# Autodesk Inventor assembly: BREEZE-S01
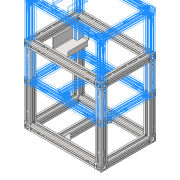
[picture p0: Inventor's stored thumbnail of the model, 180x180]
Saved by Autodesk Inventor 2020 (Build 240168000, 168)
## iProperties
Created: 2020-04-12
Part Number: BREEZE-S01
Document SubType Name: Assembly
Designer: John K
Description: FRAME ASSEMBLY
Author: John K
## Documents named in this file (9)
- C:\GrabCAD\MTL Ventilator Design\BREEZE\Subassemblies\BREEZE-S01.iam
- C:\GrabCAD\MTL Ventilator Design\BREEZE\Manufactured Parts\BREEZE-M01.ipt
- C:\GrabCAD\MTL Ventilator Design\BREEZE\Manufactured Parts\BREEZE-M03.ipt
- C:\GrabCAD\MTL Ventilator Design\BREEZE\Commercial Parts\McMaster\Frame Corner.ipt
- C:\GrabCAD\MTL Ventilator Design\BREEZE\Commercial Parts\McMaster\Frame Bracket.ipt
- C:\GrabCAD\MTL Ventilator Design\BREEZE\Manufactured Parts\BREEZE-M04.ipt
- C:\GrabCAD\MTL Ventilator Design\BREEZE\Commercial Parts\McMaster\M5x14mm Button.ipt
- C:\GrabCAD\MTL Ventilator Design\BREEZE\Commercial Parts\McMaster\M5 T-Slot Fastener.ipt
- C:\GrabCAD\MTL Ventilator Design\BREEZE\Commercial Parts\McMaster\M5x8mm Flanged Button.ipt
## Components (104 placed, 8 different names)
1. BREEZE-M01:1 — Flush:1, Flush:2, Flush:3, Flush:4, Symmetry:1, Symmetry:2, Mate:1, Mate:2, Flush:10, Mate:3, Mate:4, Mate:5, Mate:6, Mate:7, Flush:24, Mate:10, Mate:14, Flush:74, Flush:117
2. BREEZE-M01:2 — Flush:2, Symmetry:2, Flush:5, Mate:2, Flush:26
3. BREEZE-M01:3 — Flush:3, Flush:5, Flush:6, Mate:22, Mate:24
4. BREEZE-M01:4 — Flush:4, Symmetry:1, Mate:1, Flush:6, Flush:11, Mate:8, Mate:23, Mate:25, Mate:26
5. BREEZE-M01:5 — Flush:7, Flush:8, Flush:9, Flush:10, Mate:3, Mate:4, Flush:12, Flush:13, Flush:14, Flush:25, Mate:15, Mate:17, Mate:19, Mate:43
6. BREEZE-M01:6 — Flush:7, Flush:9, Flush:11, Flush:16, Mate:20, Flush:71, Mate:40, Flush:100
7. BREEZE-M01:7 — Flush:12, Flush:13, Flush:15, Mate:5, Mate:11, Mate:13, Flush:49, Flush:85, Mate:34, Mate:36, Flush:112
8. BREEZE-M01:8 — Flush:14, Flush:15, Flush:16, Flush:70, Flush:86, Flush:113
9. BREEZE-M03:1 — Flush:17, Flush:18, Flush:19, Flush:21, Flush:23, Mate:6, Mate:7, Flush:24, Mate:8, Mate:9, Mate:12, Mate:30, Flush:84, Mate:32
10. BREEZE-M03:2 — Flush:17, Flush:21, Flush:22, Flush:26, Mate:21, Flush:48, Mate:31, Flush:88, Flush:87, Flush:93, Flush:94, Mate:37, Flush:89
11. BREEZE-M03:3 — Flush:19, Flush:20, Flush:22, Flush:47
12. BREEZE-M03:4 — Flush:18, Flush:20, Flush:23, Flush:25, Mate:16, Flush:43
13. BREEZE-M03:5 — Flush:43, Mate:17, Flush:45, Mate:18, Flush:47, Mate:38, Mate:39
14. BREEZE-M04:1 — Mate:21, Flush:48, Flush:49
15. Frame Corner:1 — Mate:9, Mate:10, Mate:11, Flush:27, Flush:28, Flush:29, Flush:30, Flush:33, Flush:34, Flush:35, Insert:1, Insert:2, Insert:3
16. Frame Corner:2 — Flush:27, Flush:30, Flush:31, Mate:13, Insert:4, Insert:5, Insert:6
17. Frame Corner:3 — Flush:29, Flush:31, Flush:32, Insert:7, Insert:8, Insert:9
18. Frame Corner:4 — Flush:28, Flush:32, Flush:33, Mate:12, Insert:10, Insert:11, Insert:12
19. Frame Corner:5 — Flush:34, Flush:35, Mate:14, Flush:36, Flush:37, Flush:39, Flush:40, Flush:42, Insert:13, Insert:14, Insert:15
20. Frame Corner:6 — Flush:36, Flush:37, Mate:15, Flush:38, Insert:16, Insert:17, Insert:18
21. Frame Corner:7 — Flush:38, Flush:39, Flush:41, Insert:19, Insert:20, Insert:21
22. Frame Corner:8 — Flush:40, Flush:41, Flush:42, Mate:16, Insert:22, Insert:23, Insert:24
23. Frame Bracket:1 — Flush:44, Flush:45, Flush:46, Mate:18, Mate:20, Mate:41, Mate:42
24. Frame Bracket:2 — Flush:44, Flush:46, Mate:19
25. M5 T-Slot Fastener:48 — Flush:112, Flush:114, Flush:115, Flush:116, Flush:117
26. M5 T-Slot Fastener:49 — Flush:113, Flush:114, Flush:115
27. M5x14mm Button:1 — Insert:1
28. M5x14mm Button:2 — Insert:2
29. M5x14mm Button:3 — Insert:3
30. M5x14mm Button:4 — Insert:4
31. M5x14mm Button:5 — Insert:5
32. M5x14mm Button:6 — Insert:6
33. M5x14mm Button:7 — Insert:7
34. M5x14mm Button:8 — Insert:8
35. M5x14mm Button:9 — Insert:9
36. M5x14mm Button:10 — Insert:10
37. M5x14mm Button:11 — Insert:11
38. M5x14mm Button:12 — Insert:12
39. M5x14mm Button:13 — Insert:13
40. M5x14mm Button:14 — Insert:14
41. M5x14mm Button:15 — Insert:15
42. M5x14mm Button:16 — Insert:16
43. M5x14mm Button:17 — Insert:17
44. M5x14mm Button:18 — Insert:18
45. M5x14mm Button:19 — Insert:19
46. M5x14mm Button:20 — Insert:20
47. M5x14mm Button:21 — Insert:21
48. M5x14mm Button:22 — Insert:22
49. M5x14mm Button:23 — Insert:23
50. M5x14mm Button:24 — Insert:24
51. M5 T-Slot Fastener:37 — Flush:90, Flush:91, Flush:92, Mate:33, Flush:93, Mate:35, Flush:94, Mate:37, Insert:25
52. M5 T-Slot Fastener:38 — Flush:90, Mate:34, Mate:36, Insert:27, Flush:116
53. M5 T-Slot Fastener:39 — Flush:91, Flush:92, Mate:33, Mate:35, Insert:26
54. M5x8mm Flanged Button:1 — Insert:25
55. M5x8mm Flanged Button:2 — Insert:26
56. M5x8mm Flanged Button:3 — Insert:27
57. M5 T-Slot Fastener:40 — Flush:98, Mate:43, Flush:99, Insert:28
58. M5 T-Slot Fastener:41 — Flush:95, Flush:96, Symmetry:6, Insert:29
59. M5 T-Slot Fastener:42 — Flush:95, Flush:96, Flush:97, Flush:98, Mate:38, Symmetry:6, Mate:39, Mate:42, Insert:30
60. M5 T-Slot Fastener:43 — Flush:97, Mate:40, Mate:41, Flush:99, Insert:31
61. M5x8mm Flanged Button:4 — Insert:28
62. M5x8mm Flanged Button:5 — Insert:29
63. M5x8mm Flanged Button:6 — Insert:30
64. M5x8mm Flanged Button:7 — Insert:31
65. M5 T-Slot Fastener:44 — Flush:101, Flush:102, Flush:111
66. M5 T-Slot Fastener:45 — Flush:103, Flush:104, Flush:110
67. M5 T-Slot Fastener:46 — Flush:105, Flush:107, Mate:44, Flush:111
68. M5 T-Slot Fastener:47 — Flush:106, Flush:108, Flush:109, Flush:110
69. M5 T-Slot Fastener:1 — Flush:55, Flush:61, Flush:65, Flush:66, Mate:22, Mate:24, Flush:87
70. M5 T-Slot Fastener:12 — Flush:64, Flush:65, Flush:69, Flush:70, Flush:88, Symmetry:4
71. M5 T-Slot Fastener:9 — Flush:60, Flush:64, Flush:68, Symmetry:4
72. M5 T-Slot Fastener:2 — Flush:59, Flush:60, Flush:63, Flush:66, Mate:23, Flush:75
73. M5 T-Slot Fastener:8 — Flush:58, Flush:59, Flush:63, Flush:67, Flush:76
74. M5 T-Slot Fastener:10 — Flush:57, Flush:58, Flush:62, Flush:68
75. M5 T-Slot Fastener:11 — Flush:56, Flush:57, Flush:62, Flush:69, Flush:71
76. M5 T-Slot Fastener:7 — Flush:55, Flush:56, Flush:61, Flush:67, Flush:100
77. M5 T-Slot Fastener:3 — Flush:50, Flush:54, Flush:72, Mate:25, Mate:26, Flush:75
78. M5 T-Slot Fastener:4 — Flush:52, Flush:53, Flush:72, Flush:74
79. M5 T-Slot Fastener:6 — Flush:51, Flush:52, Flush:53, Flush:73
80. M5 T-Slot Fastener:5 — Flush:50, Flush:51, Flush:54, Flush:73, Flush:76
81. M5 T-Slot Fastener:19
82. M5 T-Slot Fastener:20
83. M5 T-Slot Fastener:21
84. M5 T-Slot Fastener:22
85. M5 T-Slot Fastener:23
86. M5 T-Slot Fastener:24
87. M5 T-Slot Fastener:25
88. M5 T-Slot Fastener:26
89. M5 T-Slot Fastener:27
90. M5 T-Slot Fastener:28
91. M5 T-Slot Fastener:29
92. M5 T-Slot Fastener:30
93. M5 T-Slot Fastener:14 — Flush:78, Flush:79, Mate:28, Flush:82, Flush:89, Symmetry:5
94. M5 T-Slot Fastener:16 — Flush:79, Flush:80, Mate:28, Flush:83, Flush:86, Symmetry:5
95. M5 T-Slot Fastener:17 — Flush:81, Mate:27, Flush:83, Flush:85
96. M5 T-Slot Fastener:15 — Flush:77, Flush:78, Mate:29, Mate:30, Flush:84, Mate:32, Flush:105, Flush:106, Flush:107, Flush:108, Flush:109, Mate:44
97. M5 T-Slot Fastener:13 — Flush:77, Mate:27, Flush:82
98. M5 T-Slot Fastener:18 — Flush:80, Flush:81, Mate:29, Mate:31, Flush:101, Flush:102, Flush:103, Flush:104
99. M5 T-Slot Fastener:31
100. M5 T-Slot Fastener:32
101. M5 T-Slot Fastener:33
102. M5 T-Slot Fastener:34
103. M5 T-Slot Fastener:35
104. M5 T-Slot Fastener:36
## Component patterns: (2 elements, first: M5 T-Slot Fastener:1 + M5 T-Slot Fastener:12 + M5 T-Slot Fastener:9 + M5 T-Slot Fastener:2 + M5 T-Slot Fastener:8 + M5 T-Slot Fastener:10 + M5 T-Slot Fastener:11 + M5 T-Slot Fastener:7 + M5 T-Slot Fastener:3 + M5 T-Slot Fastener:4 + M5 T-Slot Fastener:6 + M5 T-Slot Fastener:5), (2 elements, first: M5 T-Slot Fastener:14 + M5 T-Slot Fastener:16 + M5 T-Slot Fastener:17 + M5 T-Slot Fastener:15 + M5 T-Slot Fastener:13 + M5 T-Slot Fastener:18)
## Relationships (197: Flush 117, Mate 44, Insert 31, Symmetry 5)
- Flush:1: BREEZE-M01:1
- Flush:2: BREEZE-M01:1 ↔ BREEZE-M01:2
- Flush:3: BREEZE-M01:1 ↔ BREEZE-M01:3
- Flush:4: BREEZE-M01:1 ↔ BREEZE-M01:4
- Symmetry:1: BREEZE-M01:1 ↔ BREEZE-M01:4
- Symmetry:2: BREEZE-M01:1 ↔ BREEZE-M01:2
- Mate:1: BREEZE-M01:1 ↔ BREEZE-M01:4
- Flush:5: BREEZE-M01:2 ↔ BREEZE-M01:3
- Mate:2: BREEZE-M01:1 ↔ BREEZE-M01:2
- Flush:6: BREEZE-M01:3 ↔ BREEZE-M01:4
- Flush:7: BREEZE-M01:5 ↔ BREEZE-M01:6
- Flush:8: BREEZE-M01:5
- Flush:9: BREEZE-M01:5 ↔ BREEZE-M01:6
- Flush:10: BREEZE-M01:1 ↔ BREEZE-M01:5
- Flush:11: BREEZE-M01:4 ↔ BREEZE-M01:6
- Mate:3: BREEZE-M01:1 ↔ BREEZE-M01:5
- Mate:4: BREEZE-M01:1 ↔ BREEZE-M01:5
- Flush:12: BREEZE-M01:5 ↔ BREEZE-M01:7
- Flush:13: BREEZE-M01:5 ↔ BREEZE-M01:7
- Flush:14: BREEZE-M01:5 ↔ BREEZE-M01:8
- Flush:15: BREEZE-M01:7 ↔ BREEZE-M01:8
- Mate:5: BREEZE-M01:1 ↔ BREEZE-M01:7
- Flush:16: BREEZE-M01:6 ↔ BREEZE-M01:8
- Flush:17: BREEZE-M03:1 ↔ BREEZE-M03:2
- Flush:18: BREEZE-M03:1 ↔ BREEZE-M03:4
- Flush:19: BREEZE-M03:1 ↔ BREEZE-M03:3
- Flush:20: BREEZE-M03:3 ↔ BREEZE-M03:4
- Flush:21: BREEZE-M03:1 ↔ BREEZE-M03:2
- Flush:22: BREEZE-M03:2 ↔ BREEZE-M03:3
- Flush:23: BREEZE-M03:1 ↔ BREEZE-M03:4
- Mate:6: BREEZE-M01:1 ↔ BREEZE-M03:1
- Mate:7: BREEZE-M01:1 ↔ BREEZE-M03:1
- Flush:24: BREEZE-M01:1 ↔ BREEZE-M03:1
- Flush:25: BREEZE-M01:5 ↔ BREEZE-M03:4
- Flush:26: BREEZE-M01:2 ↔ BREEZE-M03:2
- Mate:8: BREEZE-M01:4 ↔ BREEZE-M03:1
- Mate:9: BREEZE-M03:1 ↔ Frame Corner:1
- Mate:10: BREEZE-M01:1 ↔ Frame Corner:1
- Mate:11: BREEZE-M01:7 ↔ Frame Corner:1
- Flush:27: Frame Corner:1 ↔ Frame Corner:2
- Flush:28: Frame Corner:1 ↔ Frame Corner:4
- Flush:29: Frame Corner:1 ↔ Frame Corner:3
- Flush:30: Frame Corner:1 ↔ Frame Corner:2
- Flush:31: Frame Corner:2 ↔ Frame Corner:3
- Flush:32: Frame Corner:3 ↔ Frame Corner:4
- Flush:33: Frame Corner:1 ↔ Frame Corner:4
- Mate:12: BREEZE-M03:1 ↔ Frame Corner:4
- Mate:13: BREEZE-M01:7 ↔ Frame Corner:2
- Flush:34: Frame Corner:1 ↔ Frame Corner:5
- Flush:35: Frame Corner:1 ↔ Frame Corner:5
- Mate:14: BREEZE-M01:1 ↔ Frame Corner:5
- Flush:36: Frame Corner:5 ↔ Frame Corner:6
- Flush:37: Frame Corner:5 ↔ Frame Corner:6
- Mate:15: BREEZE-M01:5 ↔ Frame Corner:6
- Flush:38: Frame Corner:6 ↔ Frame Corner:7
- Flush:39: Frame Corner:5 ↔ Frame Corner:7
- Flush:40: Frame Corner:5 ↔ Frame Corner:8
- Flush:41: Frame Corner:7 ↔ Frame Corner:8
- Flush:42: Frame Corner:5 ↔ Frame Corner:8
- Mate:16: BREEZE-M03:4 ↔ Frame Corner:8
- Flush:43: BREEZE-M03:4 ↔ BREEZE-M03:5
- Mate:17: BREEZE-M01:5 ↔ BREEZE-M03:5
- Flush:44: Frame Bracket:1 ↔ Frame Bracket:2
- Flush:45: BREEZE-M03:5 ↔ Frame Bracket:1
- Flush:46: Frame Bracket:1 ↔ Frame Bracket:2
- Mate:18: BREEZE-M03:5 ↔ Frame Bracket:1
- Mate:19: BREEZE-M01:5 ↔ Frame Bracket:2
- Mate:20: BREEZE-M01:6 ↔ Frame Bracket:1
- Flush:47 (-84.308 mm): BREEZE-M03:3 ↔ BREEZE-M03:5
- Mate:21: BREEZE-M03:2 ↔ BREEZE-M04:1
- Flush:48 (1 mm): BREEZE-M03:2 ↔ BREEZE-M04:1
- Flush:49 (1 mm): BREEZE-M01:7 ↔ BREEZE-M04:1
- Insert:1: Frame Corner:1 ↔ M5x14mm Button:1
- Insert:2: Frame Corner:1 ↔ M5x14mm Button:2
- Insert:3: Frame Corner:1 ↔ M5x14mm Button:3
- Insert:4: Frame Corner:2 ↔ M5x14mm Button:4
- Insert:5: Frame Corner:2 ↔ M5x14mm Button:5
- Insert:6: Frame Corner:2 ↔ M5x14mm Button:6
- Insert:7: Frame Corner:3 ↔ M5x14mm Button:7
- Insert:8: Frame Corner:3 ↔ M5x14mm Button:8
- Insert:9: Frame Corner:3 ↔ M5x14mm Button:9
- Insert:10: Frame Corner:4 ↔ M5x14mm Button:10
- Insert:11: Frame Corner:4 ↔ M5x14mm Button:11
- Insert:12: Frame Corner:4 ↔ M5x14mm Button:12
- Insert:13: Frame Corner:5 ↔ M5x14mm Button:13
- Insert:14: Frame Corner:5 ↔ M5x14mm Button:14
- Insert:15: Frame Corner:5 ↔ M5x14mm Button:15
- Insert:16: Frame Corner:6 ↔ M5x14mm Button:16
- Insert:17: Frame Corner:6 ↔ M5x14mm Button:17
- Insert:18: Frame Corner:6 ↔ M5x14mm Button:18
- Insert:19: Frame Corner:7 ↔ M5x14mm Button:19
- Insert:20: Frame Corner:7 ↔ M5x14mm Button:20
- Insert:21: Frame Corner:7 ↔ M5x14mm Button:21
- Insert:22: Frame Corner:8 ↔ M5x14mm Button:22
- Insert:23: Frame Corner:8 ↔ M5x14mm Button:23
- Insert:24: Frame Corner:8 ↔ M5x14mm Button:24
- Flush:50: M5 T-Slot Fastener:3 ↔ M5 T-Slot Fastener:5
- Flush:51: M5 T-Slot Fastener:6 ↔ M5 T-Slot Fastener:5
- Flush:52: M5 T-Slot Fastener:4 ↔ M5 T-Slot Fastener:6
- Flush:53: M5 T-Slot Fastener:4 ↔ M5 T-Slot Fastener:6
- Flush:54: M5 T-Slot Fastener:3 ↔ M5 T-Slot Fastener:5
- Flush:55: M5 T-Slot Fastener:1 ↔ M5 T-Slot Fastener:7
- Flush:56: M5 T-Slot Fastener:11 ↔ M5 T-Slot Fastener:7
- Flush:57: M5 T-Slot Fastener:10 ↔ M5 T-Slot Fastener:11
- Flush:58: M5 T-Slot Fastener:8 ↔ M5 T-Slot Fastener:10
- Flush:59: M5 T-Slot Fastener:2 ↔ M5 T-Slot Fastener:8
- Flush:60: M5 T-Slot Fastener:9 ↔ M5 T-Slot Fastener:2
- Flush:61: M5 T-Slot Fastener:1 ↔ M5 T-Slot Fastener:7
- Flush:62: M5 T-Slot Fastener:10 ↔ M5 T-Slot Fastener:11
- Flush:63: M5 T-Slot Fastener:2 ↔ M5 T-Slot Fastener:8
- Flush:64: M5 T-Slot Fastener:12 ↔ M5 T-Slot Fastener:9
- Flush:65: M5 T-Slot Fastener:1 ↔ M5 T-Slot Fastener:12
- Flush:66: M5 T-Slot Fastener:1 ↔ M5 T-Slot Fastener:2
- Flush:67: M5 T-Slot Fastener:8 ↔ M5 T-Slot Fastener:7
- Flush:68: M5 T-Slot Fastener:9 ↔ M5 T-Slot Fastener:10
- Flush:69: M5 T-Slot Fastener:12 ↔ M5 T-Slot Fastener:11
- Flush:70: BREEZE-M01:8 ↔ M5 T-Slot Fastener:12
- Mate:22: BREEZE-M01:3 ↔ M5 T-Slot Fastener:1
- Mate:23: BREEZE-M01:4 ↔ M5 T-Slot Fastener:2
- Flush:71: BREEZE-M01:6 ↔ M5 T-Slot Fastener:11
- Mate:24: BREEZE-M01:3 ↔ M5 T-Slot Fastener:1
- Flush:72: M5 T-Slot Fastener:3 ↔ M5 T-Slot Fastener:4
- Flush:73: M5 T-Slot Fastener:6 ↔ M5 T-Slot Fastener:5
- Mate:25: BREEZE-M01:4 ↔ M5 T-Slot Fastener:3
- Flush:74: BREEZE-M01:1 ↔ M5 T-Slot Fastener:4
- Mate:26: BREEZE-M01:4 ↔ M5 T-Slot Fastener:3
- Flush:75: M5 T-Slot Fastener:2 ↔ M5 T-Slot Fastener:3
- Flush:76: M5 T-Slot Fastener:8 ↔ M5 T-Slot Fastener:5
- Flush:77: M5 T-Slot Fastener:15 ↔ M5 T-Slot Fastener:13
- Flush:78: M5 T-Slot Fastener:14 ↔ M5 T-Slot Fastener:15
- Flush:79: M5 T-Slot Fastener:14 ↔ M5 T-Slot Fastener:16
- Flush:80: M5 T-Slot Fastener:16 ↔ M5 T-Slot Fastener:18
- Flush:81: M5 T-Slot Fastener:17 ↔ M5 T-Slot Fastener:18
- Mate:27: M5 T-Slot Fastener:17 ↔ M5 T-Slot Fastener:13
- Mate:28: M5 T-Slot Fastener:14 ↔ M5 T-Slot Fastener:16
- Mate:29: M5 T-Slot Fastener:15 ↔ M5 T-Slot Fastener:18
- Flush:82: M5 T-Slot Fastener:14 ↔ M5 T-Slot Fastener:13
- Flush:83: M5 T-Slot Fastener:16 ↔ M5 T-Slot Fastener:17
- Mate:30: BREEZE-M03:1 ↔ M5 T-Slot Fastener:15
- Flush:84: BREEZE-M03:1 ↔ M5 T-Slot Fastener:15
- Mate:31: BREEZE-M03:2 ↔ M5 T-Slot Fastener:18
- Flush:85: BREEZE-M01:7 ↔ M5 T-Slot Fastener:17
- Flush:86: BREEZE-M01:8 ↔ M5 T-Slot Fastener:16
- Mate:32: BREEZE-M03:1 ↔ M5 T-Slot Fastener:15
- Flush:87 (35.63 mm): BREEZE-M03:2 ↔ M5 T-Slot Fastener:1
- Flush:88 (46.947 mm): BREEZE-M03:2 ↔ M5 T-Slot Fastener:12
- Symmetry:4: M5 T-Slot Fastener:12 ↔ M5 T-Slot Fastener:9
- Flush:89 (52 mm): BREEZE-M03:2 ↔ M5 T-Slot Fastener:14
- Symmetry:5: M5 T-Slot Fastener:14 ↔ M5 T-Slot Fastener:16
- Flush:90: M5 T-Slot Fastener:37 ↔ M5 T-Slot Fastener:38
- Flush:91: M5 T-Slot Fastener:37 ↔ M5 T-Slot Fastener:39
- Flush:92: M5 T-Slot Fastener:37 ↔ M5 T-Slot Fastener:39
- Mate:33: M5 T-Slot Fastener:37 ↔ M5 T-Slot Fastener:39
- Flush:93: BREEZE-M03:2 ↔ M5 T-Slot Fastener:37
- Mate:34: BREEZE-M01:7 ↔ M5 T-Slot Fastener:38
- Mate:35 (-43 mm): M5 T-Slot Fastener:37 ↔ M5 T-Slot Fastener:39
- Flush:94 (29 mm): BREEZE-M03:2 ↔ M5 T-Slot Fastener:37
- Mate:36 (-23.5 mm): BREEZE-M01:7 ↔ M5 T-Slot Fastener:38
- Mate:37: BREEZE-M03:2 ↔ M5 T-Slot Fastener:37
- Insert:25 (3.8 mm): M5 T-Slot Fastener:37 ↔ M5x8mm Flanged Button:1
- Insert:26 (3.8 mm): M5 T-Slot Fastener:39 ↔ M5x8mm Flanged Button:2
- Insert:27 (3.8 mm): M5 T-Slot Fastener:38 ↔ M5x8mm Flanged Button:3
- Flush:95: M5 T-Slot Fastener:41 ↔ M5 T-Slot Fastener:42
- Flush:96: M5 T-Slot Fastener:41 ↔ M5 T-Slot Fastener:42
- Flush:97: M5 T-Slot Fastener:42 ↔ M5 T-Slot Fastener:43
- Flush:98: M5 T-Slot Fastener:40 ↔ M5 T-Slot Fastener:42
- Mate:38: BREEZE-M03:5 ↔ M5 T-Slot Fastener:42
- Symmetry:6: M5 T-Slot Fastener:41 ↔ M5 T-Slot Fastener:42
- Mate:39: BREEZE-M03:5 ↔ M5 T-Slot Fastener:42
- Mate:40: BREEZE-M01:6 ↔ M5 T-Slot Fastener:43
- Mate:41 (3.5 mm): Frame Bracket:1 ↔ M5 T-Slot Fastener:43
- Mate:42 (3.5 mm): Frame Bracket:1 ↔ M5 T-Slot Fastener:42
- Mate:43: BREEZE-M01:5 ↔ M5 T-Slot Fastener:40
- Flush:99: M5 T-Slot Fastener:40 ↔ M5 T-Slot Fastener:43
- Insert:28 (4.8 mm): M5 T-Slot Fastener:40 ↔ M5x8mm Flanged Button:4
- Insert:29 (4.8 mm): M5 T-Slot Fastener:41 ↔ M5x8mm Flanged Button:5
- Insert:30 (4.8 mm): M5 T-Slot Fastener:42 ↔ M5x8mm Flanged Button:6
- Insert:31 (4.8 mm): M5 T-Slot Fastener:43 ↔ M5x8mm Flanged Button:7
- Flush:100 (42.67 mm): BREEZE-M01:6 ↔ M5 T-Slot Fastener:7
- Flush:101: M5 T-Slot Fastener:44 ↔ M5 T-Slot Fastener:18
- Flush:102: M5 T-Slot Fastener:44 ↔ M5 T-Slot Fastener:18
- Flush:103: M5 T-Slot Fastener:45 ↔ M5 T-Slot Fastener:18
- Flush:104: M5 T-Slot Fastener:45 ↔ M5 T-Slot Fastener:18
- Flush:105: M5 T-Slot Fastener:46 ↔ M5 T-Slot Fastener:15
- Flush:106: M5 T-Slot Fastener:47 ↔ M5 T-Slot Fastener:15
- Flush:107: M5 T-Slot Fastener:46 ↔ M5 T-Slot Fastener:15
- Flush:108: M5 T-Slot Fastener:47 ↔ M5 T-Slot Fastener:15
- Flush:109 (46.831 mm): M5 T-Slot Fastener:47 ↔ M5 T-Slot Fastener:15
- Mate:44 (-46.831 mm): M5 T-Slot Fastener:46 ↔ M5 T-Slot Fastener:15
- Flush:110: M5 T-Slot Fastener:45 ↔ M5 T-Slot Fastener:47
- Flush:111: M5 T-Slot Fastener:44 ↔ M5 T-Slot Fastener:46
- Flush:112: BREEZE-M01:7 ↔ M5 T-Slot Fastener:48
- Flush:113: BREEZE-M01:8 ↔ M5 T-Slot Fastener:49
- Flush:114: M5 T-Slot Fastener:48 ↔ M5 T-Slot Fastener:49
- Flush:115: M5 T-Slot Fastener:48 ↔ M5 T-Slot Fastener:49
- Flush:116: M5 T-Slot Fastener:48 ↔ M5 T-Slot Fastener:38
- Flush:117 (-19.55 mm): BREEZE-M01:1 ↔ M5 T-Slot Fastener:48
